# Autodesk Inventor assembly: frame_base_assembly
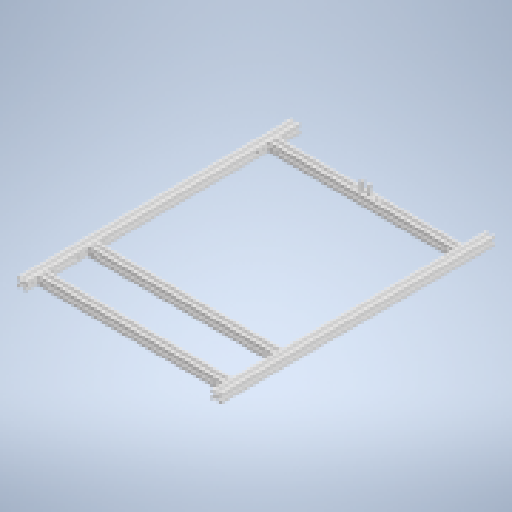
[picture p0: Inventor's stored thumbnail of the model, 512x512]
Saved by Autodesk Inventor 2024.2 (Build 282272000, 272)
## iProperties
Created: 2020-03-16
Part Number: frame_base_assembly
Document SubType Name: Assembly
Designer: Micha
Author: Micha
Revision Number: ANY
## Documents named in this file (4)
- C:\Users\Micha\Documents\493\project\jubilee_snapshot_mar_16_2020\frame_base_assembly.iam
- C:\Users\Micha\Documents\493\project\jubilee_snapshot_mar_16_2020\409mm_2020_tslot_extrusion.ipt
- C:\Users\Micha\Documents\493\project\jubilee_snapshot_mar_16_2020\604mm_2020_tslot_extrusion.ipt
- C:\Users\Micha\Documents\493\project\jubilee_snapshot_mar_16_2020\inside_hidden_corner_bracket.ipt
## Components (19 placed, 19 different names)
1. 409mm_2020_tslot_extrusion_748 — Flush:3, Flush:4, Mate:2
2. 604mm_2020_tslot_extrusion_749 — Mate:1, Flush:1, Flush:2, Flush:3, Flush:4, Mate:2, Flush:5, Flush:6, Mate:3, Mate:5, Flush:7, Flush:9, Flush:12
3. 409mm_2020_tslot_extrusion_750 — Mate:4, Mate:5, Flush:7, Flush:8, Flush:10, Flush:11, Flush:13, Flush:14, Flush:15, Flush:17, Flush:18
4. 409mm_2020_tslot_extrusion_752 — Flush:5, Flush:6, Mate:3, Mate:4
5. 604mm_2020_tslot_extrusion_753 — Mate:1, Flush:1, Flush:2, Flush:16, Flush:19
6. inside_hidden_corner_bracket_754
7. inside_hidden_corner_bracket_755
8. inside_hidden_corner_bracket_756 — Flush:8, Flush:9, Flush:10
9. inside_hidden_corner_bracket_757 — Flush:11, Flush:12, Flush:13
10. inside_hidden_corner_bracket_760
11. inside_hidden_corner_bracket_761
12. inside_hidden_corner_bracket_762
13. inside_hidden_corner_bracket_763
14. inside_hidden_corner_bracket_766 — Flush:17, Flush:18, Flush:19
15. inside_hidden_corner_bracket_767 — Flush:14, Flush:15, Flush:16
16. inside_hidden_corner_bracket_768
17. inside_hidden_corner_bracket_769
18. inside_hidden_corner_bracket_770
19. inside_hidden_corner_bracket_771
## Relationships (24: Flush 19, Mate 5)
- Mate:1 (409 mm): 604mm_2020_tslot_extrusion_749 ↔ 604mm_2020_tslot_extrusion_753
- Flush:1: 604mm_2020_tslot_extrusion_749 ↔ 604mm_2020_tslot_extrusion_753
- Flush:2: 604mm_2020_tslot_extrusion_749 ↔ 604mm_2020_tslot_extrusion_753
- Flush:3 (25 mm): 409mm_2020_tslot_extrusion_748 ↔ 604mm_2020_tslot_extrusion_749
- Flush:4: 409mm_2020_tslot_extrusion_748 ↔ 604mm_2020_tslot_extrusion_749
- Mate:2: 409mm_2020_tslot_extrusion_748 ↔ 604mm_2020_tslot_extrusion_749
- Flush:5 (50 mm): 604mm_2020_tslot_extrusion_749 ↔ 409mm_2020_tslot_extrusion_752
- Flush:6: 604mm_2020_tslot_extrusion_749 ↔ 409mm_2020_tslot_extrusion_752
- Mate:3: 604mm_2020_tslot_extrusion_749 ↔ 409mm_2020_tslot_extrusion_752
- Mate:4 (234.5 mm): 409mm_2020_tslot_extrusion_750 ↔ 409mm_2020_tslot_extrusion_752
- Mate:5: 604mm_2020_tslot_extrusion_749 ↔ 409mm_2020_tslot_extrusion_750
- Flush:7: 604mm_2020_tslot_extrusion_749 ↔ 409mm_2020_tslot_extrusion_750
- Flush:8 (7 mm): 409mm_2020_tslot_extrusion_750 ↔ inside_hidden_corner_bracket_756
- Flush:9 (-0.4 mm): 604mm_2020_tslot_extrusion_749 ↔ inside_hidden_corner_bracket_756
- Flush:10 (-0.4 mm): 409mm_2020_tslot_extrusion_750 ↔ inside_hidden_corner_bracket_756
- Flush:11 (7 mm): 409mm_2020_tslot_extrusion_750 ↔ inside_hidden_corner_bracket_757
- Flush:12 (-0.4 mm): 604mm_2020_tslot_extrusion_749 ↔ inside_hidden_corner_bracket_757
- Flush:13 (-0.4 mm): 409mm_2020_tslot_extrusion_750 ↔ inside_hidden_corner_bracket_757
- Flush:14 (7 mm): 409mm_2020_tslot_extrusion_750 ↔ inside_hidden_corner_bracket_767
- Flush:15 (-0.4 mm): 409mm_2020_tslot_extrusion_750 ↔ inside_hidden_corner_bracket_767
- Flush:16 (-0.4 mm): 604mm_2020_tslot_extrusion_753 ↔ inside_hidden_corner_bracket_767
- Flush:17 (7 mm): 409mm_2020_tslot_extrusion_750 ↔ inside_hidden_corner_bracket_766
- Flush:18 (-0.4 mm): 409mm_2020_tslot_extrusion_750 ↔ inside_hidden_corner_bracket_766
- Flush:19 (-0.4 mm): 604mm_2020_tslot_extrusion_753 ↔ inside_hidden_corner_bracket_766
